# Autodesk Inventor assembly: Assemblykadlub_demension
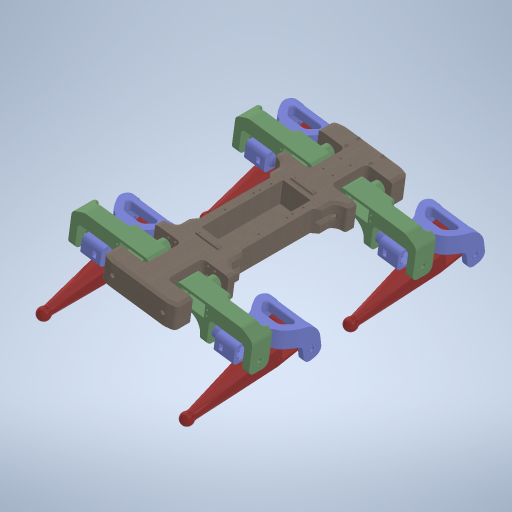
[picture p0: Inventor's stored thumbnail of the model, 512x512]
Saved by Autodesk Inventor 2023 (Build 270158000, 158)
## iProperties
Created: 2023-11-24
Part Number: Assemblykadlub_demension
Document SubType Name: Assembly
Designer: Dawid
Author: Dawid
## Documents named in this file (10)
- C:\Users\Dawid\Desktop\Robot\Github\DogRobot_MyEngineeringWork\3D_element\Assemblykadlub_demension.iam
- C:\Users\Dawid\Desktop\Robot\Github\DogRobot_MyEngineeringWork\3D_element\Kadlub1.ipt
- C:\Users\Dawid\Desktop\Robot\Github\DogRobot_MyEngineeringWork\3D_element\kadlub2.ipt
- C:\Users\Dawid\Desktop\Robot\Github\DogRobot_MyEngineeringWork\3D_element\kadlub2_f2f.ipt
- C:\Users\Dawid\Desktop\Robot\Github\DogRobot_MyEngineeringWork\3D_element\Leg1_1.ipt
- C:\Users\Dawid\Desktop\Robot\Github\DogRobot_MyEngineeringWork\3D_element\Leg1_2.ipt
- C:\Users\Dawid\Desktop\Robot\Github\DogRobot_MyEngineeringWork\3D_element\Leg1_3.ipt
- C:\Users\Dawid\Desktop\Robot\Github\DogRobot_MyEngineeringWork\3D_element\Leg1_1_MIR.ipt
- C:\Users\Dawid\Desktop\Robot\Github\DogRobot_MyEngineeringWork\3D_element\Leg1_2_MIR.ipt
- C:\Users\Dawid\Desktop\Robot\Github\DogRobot_MyEngineeringWork\3D_element\Leg1_3_MIR.ipt
## Components (15 placed, 9 different names)
1. Kadlub1:1
2. kadlub2:1
3. Leg1_1:1
4. Leg1_2:1
5. Leg1_3:1
6. Leg1_1:2
7. Leg1_2:2
8. Leg1_3:2
9. kadlub2_f2f:1
10. Leg1_1_MIR:1
11. Leg1_1_MIR:2
12. Leg1_2_MIR:1
13. Leg1_2_MIR:2
14. Leg1_3_MIR:1
15. Leg1_3_MIR:2
## Relationships (14: WeldJoint 14)
- [WeldJoint]: Kadlub1:1 ↔ kadlub2:1
- [WeldJoint]: kadlub2:1 ↔ Leg1_1:1
- [WeldJoint]: Leg1_1:1 ↔ Leg1_2:1
- [WeldJoint]: Leg1_2:1 ↔ Leg1_3:1
- [WeldJoint]: Kadlub1:1 ↔ kadlub2_f2f:1
- [WeldJoint]: Leg1_1:2 ↔ kadlub2_f2f:1
- [WeldJoint]: Leg1_1:2 ↔ Leg1_2:2
- [WeldJoint]: Leg1_2:2 ↔ Leg1_3:2
- [WeldJoint]: kadlub2:1 ↔ Leg1_1_MIR:2
- [WeldJoint]: kadlub2_f2f:1 ↔ Leg1_1_MIR:1
- [WeldJoint]: Leg1_1_MIR:1 ↔ Leg1_2_MIR:1
- [WeldJoint]: Leg1_1_MIR:2 ↔ Leg1_2_MIR:2
- [WeldJoint]: Leg1_2_MIR:1 ↔ Leg1_3_MIR:1
- [WeldJoint]: Leg1_2_MIR:2 ↔ Leg1_3_MIR:2
## Named parameters: d17_d21 = 0 mm, d18_d22 = 0 mm
